# Autodesk Inventor assembly: Controller_PCB
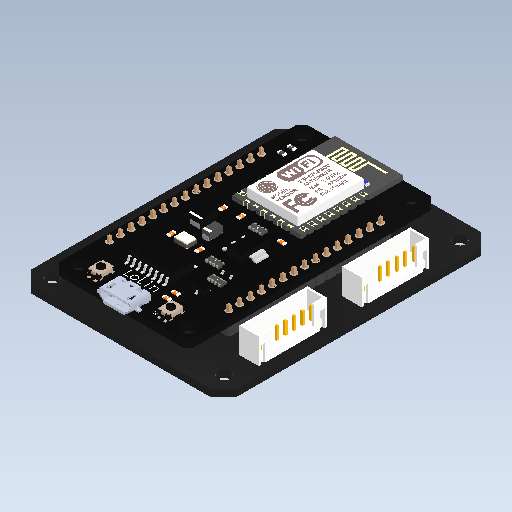
[picture p0: Inventor's stored thumbnail of the model, 512x512]
Saved by Autodesk Inventor 2020 (Build 240168000, 168)
## iProperties
Created: 2019-05-21
Part Number: Controller_PCB
Document SubType Name: Assembly
Designer: chitl
Author: chitl
## Documents named in this file (4)
- C:\Users\chitl\Desktop\OneWheel\Wheel Assembled\Electronics\Controller_PCB.iam
- C:\Users\chitl\Desktop\OneWheel\Wheel Assembled\Electronics\lolin-nodemcu-esp8266-development-board-v3-1.snapshot.3\Lolin NodeMCU ESP8266 V3.iam
- C:\Users\chitl\Desktop\OneWheel\Wheel Assembled\Electronics\jst-ph-sockets-3-to-10-pins-1.snapshot.3\JST Socket 7 Pin.iam
- C:\Users\chitl\Desktop\OneWheel\Wheel Assembled\Electronics\PCB.ipt
## Components (4 placed, 3 different names)
1. Lolin NodeMCU ESP8266 V3:1 [sub-assembly] — Mate:3
2. JST Socket 7 Pin:1 [sub-assembly] — Mate:2
3. JST Socket 7 Pin:2 [sub-assembly] — Mate:1
4. PCB:1 — Mate:1, Mate:2, Mate:3
## Relationships (3: Mate 3)
- Mate:1: JST Socket 7 Pin:2 ↔ PCB:1
- Mate:2: JST Socket 7 Pin:1 ↔ PCB:1
- Mate:3: Lolin NodeMCU ESP8266 V3:1 ↔ PCB:1
